# Autodesk Inventor assembly: 900-50-PROFILES-ANGLE-CONN-20x20-01
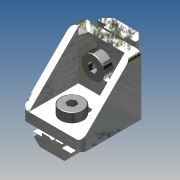
[picture p0: Inventor's stored thumbnail of the model, 180x180]
Saved by Autodesk Inventor 2018.2 (Build 222227000, 227)
## iProperties
Manager: feesmrt
Company: FRANCOR
Part Number: 900-50-PROFILES-ANGLE-CONN-20x20-01
Project: Rescue Robot
Cost Center: -
Material: Generisch
Document SubType Name: Assembly
Designer: feesmrt
Engineer: feesmrt
Authority: feesmrt
Subject: Rescue Robot
Author: feesmrt
Revision Number: 1
## Documents named in this file (4)
- D:\Programmierung\FRANC0R\CAD\02-Rocker-Bogie-Robot\900-COMPONENTS\900-50-PROFILES\900-50-PROFILES-ANGLE-CONN-20x20-01.iam
- D:\Programmierung\FRANC0R\CAD\02-Rocker-Bogie-Robot\900-COMPONENTS\900-50-PROFILES\900-50-PROFILES-ANGLE-CONN-20x20.ipt
- D:\Programmierung\FRANC0R\CAD\02-Rocker-Bogie-Robot\900-COMPONENTS\900-40-SCREWS\900-40-SCREWS-DIN7984_M4x8.ipt
- D:\Programmierung\FRANC0R\CAD\02-Rocker-Bogie-Robot\900-COMPONENTS\900-50-PROFILES\900-50-PROFILES-CONN-N6xM4.ipt
## Components (5 placed, 3 different names)
1. 900-50-PROFILES-ANGLE-CONN-20x20:1 — Passend:1, Passend:2, Passend:3, Passend:4, Passend:9, Passend:10
2. 900-40-SCREWS-DIN7984_M4x8:1 — Passend:1, Passend:4, Passend:6, Passend:8
3. 900-40-SCREWS-DIN7984_M4x8:2 — Passend:2, Passend:3, Passend:5, Passend:7
4. 900-50-PROFILES-CONN-N6xM4:1 — Passend:8, Passend:9, Passend:11
5. 900-50-PROFILES-CONN-N6xM4:2 — Passend:7, Passend:10, Passend:12
## Relationships (12: Mate 12)
- Passend:1 [Mate]: 900-50-PROFILES-ANGLE-CONN-20x20:1 ↔ 900-40-SCREWS-DIN7984_M4x8:1
- Passend:2 [Mate]: 900-50-PROFILES-ANGLE-CONN-20x20:1 ↔ 900-40-SCREWS-DIN7984_M4x8:2
- Passend:3 [Mate] (-12 mm): 900-50-PROFILES-ANGLE-CONN-20x20:1 ↔ 900-40-SCREWS-DIN7984_M4x8:2
- Passend:4 [Mate] (-12 mm): 900-50-PROFILES-ANGLE-CONN-20x20:1 ↔ 900-40-SCREWS-DIN7984_M4x8:1
- Passend:5 [Mate]: 900-40-SCREWS-DIN7984_M4x8:2
- Passend:6 [Mate]: 900-40-SCREWS-DIN7984_M4x8:1
- Passend:7 [Mate]: 900-40-SCREWS-DIN7984_M4x8:2 ↔ 900-50-PROFILES-CONN-N6xM4:2
- Passend:8 [Mate]: 900-40-SCREWS-DIN7984_M4x8:1 ↔ 900-50-PROFILES-CONN-N6xM4:1
- Passend:9 [Mate] (1.5 mm): 900-50-PROFILES-ANGLE-CONN-20x20:1 ↔ 900-50-PROFILES-CONN-N6xM4:1
- Passend:10 [Mate] (1.5 mm): 900-50-PROFILES-ANGLE-CONN-20x20:1 ↔ 900-50-PROFILES-CONN-N6xM4:2
- Passend:11 [Mate]: 900-50-PROFILES-CONN-N6xM4:1
- Passend:12 [Mate]: 900-50-PROFILES-CONN-N6xM4:2
